# Autodesk Inventor assembly: ServoBlock
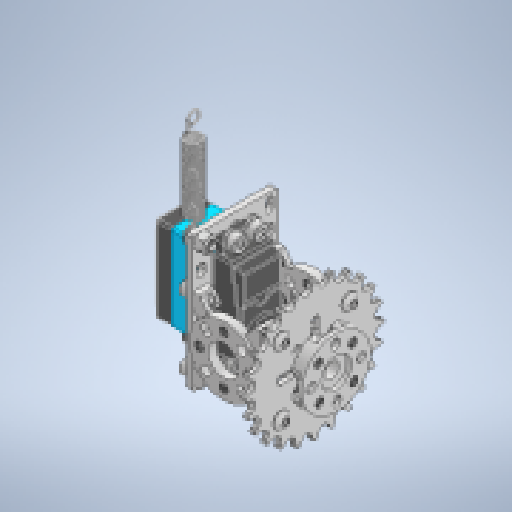
[picture p0: Inventor's stored thumbnail of the model, 512x512]
Saved by Autodesk Inventor 2023 (Build 270158000, 158)
## iProperties
Created: 2022-09-10
Part Number: ServoBlock
Document SubType Name: Assembly
Designer: deli
Author: deli
## Documents named in this file (7)
- C:\Users\deli\OneDrive - Eastside Preparatory School\FTC\8103-power-play\CAD\ServoBlock.iam
- C:\Users\deli\OneDrive - Eastside Preparatory School\FTC\8103-power-play\CAD\FTC-parts\DS3225-SG-Coreless.ipt
- C:\Users\deli\OneDrive - Eastside Preparatory School\FTC\8103-power-play\CAD\FTC-parts\goBILDA\3202-0001-2501.ipt
- C:\Users\deli\OneDrive - Eastside Preparatory School\FTC\8103-power-play\CAD\3311-0014-0024 with 19mm hole.ipt
- C:\Users\deli\OneDrive - Eastside Preparatory School\FTC\8103-power-play\CAD\FTC-parts\goBILDA\2802-0004-0010.ipt
- C:\Users\deli\OneDrive - Eastside Preparatory School\FTC\8103-power-play\CAD\FTC-parts\goBILDA\2915-0001-0002.ipt
- C:\Users\deli\OneDrive - Eastside Preparatory School\FTC\8103-power-play\CAD\FTC-parts\goBILDA\2812-0004-0007.ipt
## Components (10 placed, 6 different names)
1. DS3225-SG-Coreless:1 — Mate:1, Mate:2, Angle:1
2. 3202-0001-2501:1 — Mate:1, Mate:2, Angle:1, Mate:6, Mate:7, Mate:8, Mate:17, Mate:18, Mate:19, Mate:20
3. 3311-0014-0024 with 19mm hole:1 — Mate:6, Mate:7, Mate:8, Mate:11, Mate:12, Mate:13, Mate:14, Mate:15, Mate:16
4. 2802-0004-0010:1 — Mate:12
5. 2802-0004-0010:2 — Mate:15, Mate:16
6. 2802-0004-0010:3 — Mate:11, Mate:13
7. 2802-0004-0010:4 — Mate:14
8. 2915-0001-0002:1 — Mate:17, Mate:18, Mate:22
9. 2802-0004-0010:5 — Mate:19, Mate:21, Mate:22
10. 2812-0004-0007:1 — Mate:20, Mate:21
## Relationships (20: Mate 19, Angle 1)
- Mate:1: DS3225-SG-Coreless:1 ↔ 3202-0001-2501:1
- Mate:2: DS3225-SG-Coreless:1 ↔ 3202-0001-2501:1
- Angle:1 (0 deg): DS3225-SG-Coreless:1 ↔ 3202-0001-2501:1
- Mate:6: 3202-0001-2501:1 ↔ 3311-0014-0024 with 19mm hole:1
- Mate:7: 3202-0001-2501:1 ↔ 3311-0014-0024 with 19mm hole:1
- Mate:8: 3202-0001-2501:1 ↔ 3311-0014-0024 with 19mm hole:1
- [Mate]: 3311-0014-0024 with 19mm hole:1 ↔ 2802-0004-0010:4
- [Mate]: 3311-0014-0024 with 19mm hole:1 ↔ 2802-0004-0010:1
- Mate:11: 3311-0014-0024 with 19mm hole:1 ↔ 2802-0004-0010:3
- Mate:12: 3311-0014-0024 with 19mm hole:1 ↔ 2802-0004-0010:1
- Mate:13: 3311-0014-0024 with 19mm hole:1 ↔ 2802-0004-0010:3
- Mate:14: 3311-0014-0024 with 19mm hole:1 ↔ 2802-0004-0010:4
- Mate:15: 3311-0014-0024 with 19mm hole:1 ↔ 2802-0004-0010:2
- Mate:16: 3311-0014-0024 with 19mm hole:1 ↔ 2802-0004-0010:2
- Mate:17 (0.6 mm): 3202-0001-2501:1 ↔ 2915-0001-0002:1
- Mate:18: 3202-0001-2501:1 ↔ 2915-0001-0002:1
- Mate:19: 3202-0001-2501:1 ↔ 2802-0004-0010:5
- Mate:20: 3202-0001-2501:1 ↔ 2812-0004-0007:1
- Mate:21: 2802-0004-0010:5 ↔ 2812-0004-0007:1
- Mate:22 (0.6 mm): 2915-0001-0002:1 ↔ 2802-0004-0010:5
